# Autodesk Inventor assembly: Assembly6
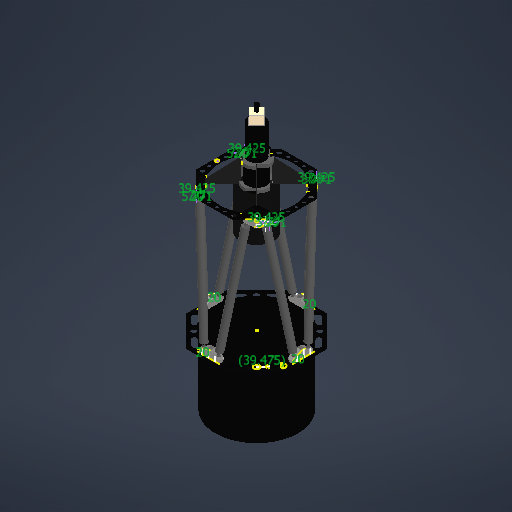
[picture p0: Inventor's stored thumbnail of the model, 512x512]
Saved by Autodesk Inventor 2026.2 (Build 302298000, 298)
## iProperties
Created: 2025-12-09
Part Number: Assembly6
Document SubType Name: Assembly
Designer: Thoma
Author: Thoma
## Documents named in this file (13)
- C:\Users\Thoma\OneDrive\Desktop\Inventor\Quarter_Open\Version_2_Flat\Main.iam
- C:\Users\Thoma\OneDrive\Desktop\Inventor\Quarter_Open\Version_2_Flat\Telescope_End.ipt
- C:\Users\Thoma\OneDrive\Desktop\Inventor\Quarter_Open\Version_2_Flat\Triangle.ipt
- C:\Users\Thoma\OneDrive\Desktop\Inventor\Quarter_Open\Version_2_Flat\Triangle_Bracket_Top.ipt
- C:\Users\Thoma\OneDrive\Desktop\Inventor\Quarter_Open\Version_2_Flat\Carbon_Fibre.ipt
- C:\Users\Thoma\OneDrive\Desktop\Inventor\Quarter_Open\Version_2_Flat\5mm Screw.ipt
- C:\Users\Thoma\OneDrive\Desktop\Inventor\Quarter_Open\Version_2_Flat\35mm_bolt.ipt
- C:\Users\Thoma\OneDrive\Desktop\Inventor\Quarter_Open\Version_2_Flat\Triangle_Bracket_Bottom_MIR.ipt
- C:\Users\Thoma\OneDrive\Desktop\Inventor\Quarter_Open\Version_2_Flat\Telescope_Base.ipt
- C:\Users\Thoma\OneDrive\Desktop\Inventor\Quarter_Open\Version_2_Flat\Bottom_End_Top.ipt
- C:\Users\Thoma\OneDrive\Desktop\Inventor\Quarter_Open\Version_2_Flat\Full_shaft_Simplify_3.ipt
- C:\Users\Thoma\OneDrive\Desktop\Inventor\Quarter_Open\Version_2_Flat\30mm_bolt.ipt
- C:\Users\Thoma\OneDrive\Desktop\Inventor\Quarter_Open\Version_2_Flat\Baffle.ipt
## Components (48 placed, 12 different names)
1. Telescope_End:1 — Mate:1, Mate:2, Angle:2, Mate:7, Mate:30, Mate:31, Angle:18, Mate:54, Mate:55, Mate:56, Mate:57, Angle:26, Angle:31, Mate:88, Mate:89, Mate:91, Flush:15, Mate:92
2. Triangle_Bracket_Top:1 — Mate:1, Mate:2, Angle:2, Mate:8, Mate:9, Angle:4, Mate:47, Angle:22, Mate:58
3. Carbon_Fibre:1 — Mate:7, Mate:11, Flush:1, Mate:12, Mate:13, Mate:14, Mate:15, Mate:22, Mate:23, Mate:24, Mate:25, Mate:32, Mate:33, Mate:34, Mate:35, Mate:42, Mate:43, Mate:44, Mate:45, Mate:62, Mate:83, Mate:87, Mate:93
4. Triangle:1 — Mate:8, Mate:9, Angle:4, Mate:11, Flush:1, Angle:5, Angle:6, Mate:46
5. 5mm Screw:1 — Mate:12, Mate:13, Angle:5
6. 5mm Screw:2 — Mate:14, Mate:15, Angle:6
7. 5mm Screw:3 — Mate:22, Mate:23, Mate:86
8. 5mm Screw:4 — Mate:24, Mate:25
9. 5mm Screw:5 — Mate:42, Mate:43
10. 5mm Screw:6 — Mate:44, Mate:45
11. Triangle_Bracket_Top:4 — Mate:28, Mate:29, Angle:15, Mate:30, Mate:31, Angle:18, Angle:24, Angle:28, Mate:60
12. Triangle:4 — Mate:28, Mate:29, Angle:15, Angle:16, Angle:17, Mate:50, Mate:51
13. 5mm Screw:7 — Angle:16, Mate:32, Mate:33
14. 5mm Screw:8 — Angle:17, Mate:34, Mate:35
15. 35mm_bolt:2 — Mate:50, Mate:51, Angle:24
16. 35mm_bolt:4 — Mate:46, Mate:47, Angle:22
17. Triangle_Bracket_Bottom_MIR:1 — Mate:54, Mate:79, Flush:12, Angle:38, Mate:80, Flush:13, Angle:39, Tangent:9, Angle:40, Angle:41
18. Triangle_Bracket_Bottom_MIR:2 — Mate:55, Mate:58, Angle:26, Tangent:4, Mate:77, Flush:10, Angle:36, Mate:78, Flush:11, Angle:37
19. Triangle_Bracket_Bottom_MIR:3 — Mate:56, Angle:28, Mate:60, Mate:73, Flush:6, Angle:32, Mate:74, Flush:7, Angle:33
20. Triangle_Bracket_Bottom_MIR:4 — Mate:57, Mate:75, Flush:8, Angle:34, Mate:76, Flush:9, Angle:35
21. Telescope_Base:1 — Mate:62, Mate:63, Mate:64, Angle:30, Angle:31, Mate:85
22. 30mm_bolt:1 — Mate:73, Flush:6, Angle:32
23. 30mm_bolt:2 — Mate:77, Flush:10, Angle:36
24. 30mm_bolt:3 — Mate:79, Flush:12, Angle:38
25. 30mm_bolt:4 — Mate:75, Flush:8, Angle:34
26. 30mm_bolt:5 — Mate:76, Flush:9, Angle:35
27. 30mm_bolt:6 — Mate:78, Flush:11, Angle:37
28. 30mm_bolt:7 — Mate:74, Flush:7, Angle:33
29. 30mm_bolt:8 — Mate:80, Flush:13, Angle:39
30. Baffle:1 — Mate:83, Mate:85
31. Triangle:6 — Mate:86, Angle:40, Mate:87
32. Triangle_Bracket_Top:5 — Mate:88, Angle:41, Mate:89, Mate:90, Flush:14, Angle:42
33. Triangle_Bracket_Top:6 — Mate:91, Flush:15, Mate:92, Mate:94, Mate:95, Mate:96, Flush:16, Angle:43
34. 30mm_bolt:9 — Mate:90, Flush:14, Angle:42
35. Triangle:7 — Mate:93, Mate:94, Mate:95
36. 35mm_bolt:5 — Mate:96, Flush:16, Angle:43
37. Full_shaft_Simplify_3:1 — Tangent:3, Tangent:4
38. Full_shaft_Simplify_3:2 — Tangent:9
39. Bottom_End_Top:1 — Mate:63, Mate:64, Angle:30, Tangent:3
40. Full_shaft_Simplify_3:3
41. Full_shaft_Simplify_3:4
42. Bottom_End_Top:2
43. Full_shaft_Simplify_3:5
44. Full_shaft_Simplify_3:6
45. Bottom_End_Top:3
46. Full_shaft_Simplify_3:7
47. Full_shaft_Simplify_3:8
48. Bottom_End_Top:4
## Component patterns: (4 elements, first: Full_shaft_Simplify_3:1 + Full_shaft_Simplify_3:2 + Bottom_End_Top:1)
## Relationships (101: Mate 60, Angle 26, Flush 12, Tangent 3)
- Mate:1: Telescope_End:1 ↔ Triangle_Bracket_Top:1
- Mate:2: Telescope_End:1 ↔ Triangle_Bracket_Top:1
- Angle:2 (0 deg): Telescope_End:1 ↔ Triangle_Bracket_Top:1
- Mate:7: Telescope_End:1 ↔ Carbon_Fibre:1
- Mate:8: Triangle_Bracket_Top:1 ↔ Triangle:1
- Mate:9: Triangle_Bracket_Top:1 ↔ Triangle:1
- Angle:4 (0 deg): Triangle_Bracket_Top:1 ↔ Triangle:1
- Mate:11: Carbon_Fibre:1 ↔ Triangle:1
- Flush:1: Carbon_Fibre:1 ↔ Triangle:1
- Mate:12: Carbon_Fibre:1 ↔ 5mm Screw:1
- Mate:13: Carbon_Fibre:1 ↔ 5mm Screw:1
- Angle:5 (0 deg): Triangle:1 ↔ 5mm Screw:1
- Mate:14: Carbon_Fibre:1 ↔ 5mm Screw:2
- Mate:15: Carbon_Fibre:1 ↔ 5mm Screw:2
- Angle:6 (0 deg): Triangle:1 ↔ 5mm Screw:2
- Mate:22: Carbon_Fibre:1 ↔ 5mm Screw:3
- Mate:23: Carbon_Fibre:1 ↔ 5mm Screw:3
- Mate:24: Carbon_Fibre:1 ↔ 5mm Screw:4
- Mate:25: Carbon_Fibre:1 ↔ 5mm Screw:4
- Mate:28: Triangle_Bracket_Top:4 ↔ Triangle:4
- Mate:29: Triangle_Bracket_Top:4 ↔ Triangle:4
- Angle:15 (0 deg): Triangle_Bracket_Top:4 ↔ Triangle:4
- Angle:16 (0 deg): Triangle:4 ↔ 5mm Screw:7
- Angle:17 (0 deg): Triangle:4 ↔ 5mm Screw:8
- Mate:30: Telescope_End:1 ↔ Triangle_Bracket_Top:4
- Mate:31: Telescope_End:1 ↔ Triangle_Bracket_Top:4
- Angle:18 (0 deg): Telescope_End:1 ↔ Triangle_Bracket_Top:4
- Mate:32: Carbon_Fibre:1 ↔ 5mm Screw:7
- Mate:33: Carbon_Fibre:1 ↔ 5mm Screw:7
- Mate:34: Carbon_Fibre:1 ↔ 5mm Screw:8
- Mate:35: Carbon_Fibre:1 ↔ 5mm Screw:8
- Mate:42: Carbon_Fibre:1 ↔ 5mm Screw:5
- Mate:43: Carbon_Fibre:1 ↔ 5mm Screw:5
- Mate:44: Carbon_Fibre:1 ↔ 5mm Screw:6
- Mate:45: Carbon_Fibre:1 ↔ 5mm Screw:6
- Mate:46: Triangle:1 ↔ 35mm_bolt:4
- Mate:47: Triangle_Bracket_Top:1 ↔ 35mm_bolt:4
- Angle:22 (0 deg): Triangle_Bracket_Top:1 ↔ 35mm_bolt:4
- Mate:50: Triangle:4 ↔ 35mm_bolt:2
- Mate:51: Triangle:4 ↔ 35mm_bolt:2
- Angle:24 (0 deg): Triangle_Bracket_Top:4 ↔ 35mm_bolt:2
- Mate:54: Telescope_End:1 ↔ Triangle_Bracket_Bottom_MIR:1
- Mate:55: Telescope_End:1 ↔ Triangle_Bracket_Bottom_MIR:2
- Mate:56: Telescope_End:1 ↔ Triangle_Bracket_Bottom_MIR:3
- Mate:57: Telescope_End:1 ↔ Triangle_Bracket_Bottom_MIR:4
- Mate:58: Triangle_Bracket_Top:1 ↔ Triangle_Bracket_Bottom_MIR:2
- Angle:26 (0 deg): Telescope_End:1 ↔ Triangle_Bracket_Bottom_MIR:2
- Angle:28 (0 deg): Triangle_Bracket_Top:4 ↔ Triangle_Bracket_Bottom_MIR:3
- Mate:60: Triangle_Bracket_Top:4 ↔ Triangle_Bracket_Bottom_MIR:3
- Mate:62: Carbon_Fibre:1 ↔ Telescope_Base:1
- Mate:63: Telescope_Base:1 ↔ Bottom_End_Top:1
- Mate:64: Telescope_Base:1 ↔ Bottom_End_Top:1
- Angle:30 (0 deg): Telescope_Base:1 ↔ Bottom_End_Top:1
- Angle:31 (0 deg): Telescope_End:1 ↔ Telescope_Base:1
- Tangent:3: Full_shaft_Simplify_3:1 ↔ Bottom_End_Top:1
- Tangent:4: Triangle_Bracket_Bottom_MIR:2 ↔ Full_shaft_Simplify_3:1
- Mate:73: Triangle_Bracket_Bottom_MIR:3 ↔ 30mm_bolt:1
- Flush:6: Triangle_Bracket_Bottom_MIR:3 ↔ 30mm_bolt:1
- Angle:32 (0 deg): Triangle_Bracket_Bottom_MIR:3 ↔ 30mm_bolt:1
- Mate:74: Triangle_Bracket_Bottom_MIR:3 ↔ 30mm_bolt:7
- Flush:7: Triangle_Bracket_Bottom_MIR:3 ↔ 30mm_bolt:7
- Angle:33 (0 deg): Triangle_Bracket_Bottom_MIR:3 ↔ 30mm_bolt:7
- Mate:75: Triangle_Bracket_Bottom_MIR:4 ↔ 30mm_bolt:4
- Flush:8: Triangle_Bracket_Bottom_MIR:4 ↔ 30mm_bolt:4
- Angle:34 (0 deg): Triangle_Bracket_Bottom_MIR:4 ↔ 30mm_bolt:4
- Mate:76: Triangle_Bracket_Bottom_MIR:4 ↔ 30mm_bolt:5
- Flush:9: Triangle_Bracket_Bottom_MIR:4 ↔ 30mm_bolt:5
- Angle:35 (0 deg): Triangle_Bracket_Bottom_MIR:4 ↔ 30mm_bolt:5
- Mate:77: Triangle_Bracket_Bottom_MIR:2 ↔ 30mm_bolt:2
- Flush:10: Triangle_Bracket_Bottom_MIR:2 ↔ 30mm_bolt:2
- Angle:36 (0 deg): Triangle_Bracket_Bottom_MIR:2 ↔ 30mm_bolt:2
- Mate:78: Triangle_Bracket_Bottom_MIR:2 ↔ 30mm_bolt:6
- Flush:11: Triangle_Bracket_Bottom_MIR:2 ↔ 30mm_bolt:6
- Angle:37 (0 deg): Triangle_Bracket_Bottom_MIR:2 ↔ 30mm_bolt:6
- Mate:79: Triangle_Bracket_Bottom_MIR:1 ↔ 30mm_bolt:3
- Flush:12: Triangle_Bracket_Bottom_MIR:1 ↔ 30mm_bolt:3
- Angle:38 (0 deg): Triangle_Bracket_Bottom_MIR:1 ↔ 30mm_bolt:3
- Mate:80: Triangle_Bracket_Bottom_MIR:1 ↔ 30mm_bolt:8
- Flush:13: Triangle_Bracket_Bottom_MIR:1 ↔ 30mm_bolt:8
- Angle:39 (0 deg): Triangle_Bracket_Bottom_MIR:1 ↔ 30mm_bolt:8
- Mate:83: Carbon_Fibre:1 ↔ Baffle:1
- Mate:85 (20 mm): Telescope_Base:1 ↔ Baffle:1
- Tangent:9: Triangle_Bracket_Bottom_MIR:1 ↔ Full_shaft_Simplify_3:2
- Mate:86: 5mm Screw:3 ↔ Triangle:6
- Angle:40 (0 deg): Triangle_Bracket_Bottom_MIR:1 ↔ Triangle:6
- Mate:87: Carbon_Fibre:1 ↔ Triangle:6
- Mate:88: Telescope_End:1 ↔ Triangle_Bracket_Top:5
- Angle:41 (0 deg): Triangle_Bracket_Bottom_MIR:1 ↔ Triangle_Bracket_Top:5
- Mate:89: Telescope_End:1 ↔ Triangle_Bracket_Top:5
- Mate:90: Triangle_Bracket_Top:5 ↔ 30mm_bolt:9
- Flush:14: Triangle_Bracket_Top:5 ↔ 30mm_bolt:9
- Angle:42 (0 deg): Triangle_Bracket_Top:5 ↔ 30mm_bolt:9
- Mate:91: Telescope_End:1 ↔ Triangle_Bracket_Top:6
- Flush:15: Telescope_End:1 ↔ Triangle_Bracket_Top:6
- Mate:92: Telescope_End:1 ↔ Triangle_Bracket_Top:6
- Mate:93: Carbon_Fibre:1 ↔ Triangle:7
- Mate:94: Triangle_Bracket_Top:6 ↔ Triangle:7
- Mate:95: Triangle_Bracket_Top:6 ↔ Triangle:7
- Mate:96: Triangle_Bracket_Top:6 ↔ 35mm_bolt:5
- Flush:16: Triangle_Bracket_Top:6 ↔ 35mm_bolt:5
- Angle:43 (0 deg): Triangle_Bracket_Top:6 ↔ 35mm_bolt:5
